# Autodesk Inventor assembly: L_Unit_SR-O
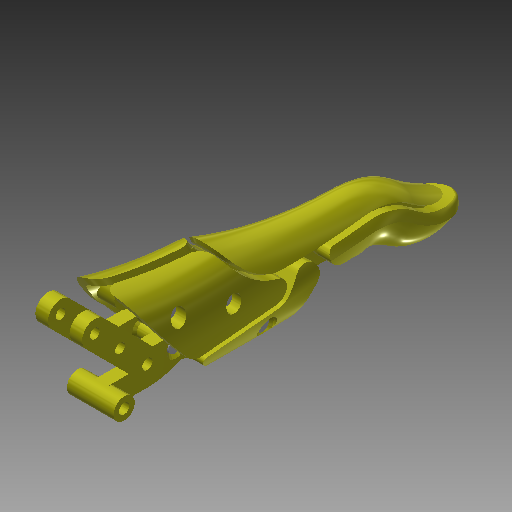
[picture p0: Inventor's stored thumbnail of the model, 512x512]
Saved by Autodesk Inventor 2018.3 (Build 223284000, 284)
## iProperties
Created: 2018-02-15
Part Number: L_Unit_SR-O
Material: 一般
Document SubType Name: Assembly
Designer: sktom
Title: Unit_SR-O
Author: sktom
## Documents named in this file (9)
- D:\CloudStrage\OneDrive\CADMech\HbSizeSMech\UnitHand\Unit_SR-H\Unit_SR-O\L_Unit_SR-O.iam
- D:\CloudStrage\OneDrive\CADMech\HbSizeSMech\UnitHand\Unit_SR-H\Unit_SR-O\L_Dummy_JointPosiion.ipt
- D:\CloudStrage\OneDrive\CADMech\HbSizeSMech\UnitHand\Unit_SR-H\Unit_SR-O\L_SR-O-01.ipt
- D:\CloudStrage\OneDrive\CADMech\HbSizeSMech\UnitHand\Unit_SR-H\Unit_SR-O\L_SR-O-02.ipt
- D:\CloudStrage\OneDrive\CADMech\HbSizeSMech\UnitHand\Unit_SR-H\Unit_SR-O\L_SR-O-03.ipt
- D:\CloudStrage\OneDrive\CADMech\HbSizeSMech\UnitHand\Unit_SR-H\Unit_SR-O\L_SR-O-04.ipt
- D:\CloudStrage\OneDrive\CADMech\HbSizeSMech\UnitHand\Unit_SR-H\Unit_SR-O\L_SR-O-05.ipt
- D:\CloudStrage\OneDrive\CADMech\HbSizeSMech\UnitHand\Unit_SR-H\Unit_SR-O\L_Parts_Shaft_Phi1.5_L6.ipt
- D:\CloudStrage\OneDrive\CADMech\HbSizeSMech\UnitHand\Unit_SR-H\Unit_SR-O\L_Parts_Screw_M1.4_L6.ipt
## Components (12 placed, 8 different names)
1. L_Dummy_JointPosiion:1 — 円柱状:3, 回転:1
2. L_SR-O-01:1 — 挿入:5, 挿入:6, 円柱状:1, 円柱状:2
3. L_SR-O-02:1 — 挿入:6, 挿入:8, 挿入:7, 回転:1
4. L_SR-O-03:1 — 挿入:2, 挿入:1, 挿入:5
5. L_SR-O-04:1 — 挿入:2, 挿入:1, 挿入:3, 挿入:4, 円柱状:3
6. L_SR-O-05:1 — 挿入:8, 挿入:7, 挿入:9, 挿入:10
7. L_Parts_Shaft_Phi1.5_L6:1 — 円柱状:1
8. L_Parts_Shaft_Phi1.5_L6:2 — 円柱状:2
9. L_Parts_Screw_M1.4_L6:1 — 挿入:4
10. L_Parts_Screw_M1.4_L6:2 — 挿入:3
11. L_Parts_Screw_M1.4_L6:3 — 挿入:9
12. L_Parts_Screw_M1.4_L6:4 — 挿入:10
## Relationships (14: Insert 10, CylindricalJoint 3, RevoluteJoint 1)
- 挿入:2 [Insert]: L_SR-O-03:1 ↔ L_SR-O-04:1
- 挿入:1 [Insert]: L_SR-O-03:1 ↔ L_SR-O-04:1
- 挿入:3 [Insert]: L_SR-O-04:1 ↔ L_Parts_Screw_M1.4_L6:2
- 挿入:4 [Insert]: L_SR-O-04:1 ↔ L_Parts_Screw_M1.4_L6:1
- 挿入:5 [Insert] (0.079 mm): L_SR-O-01:1 ↔ L_SR-O-03:1
- 挿入:6 [Insert] (0.079 mm): L_SR-O-01:1 ↔ L_SR-O-02:1
- 挿入:8 [Insert]: L_SR-O-02:1 ↔ L_SR-O-05:1
- 挿入:7 [Insert]: L_SR-O-02:1 ↔ L_SR-O-05:1
- 挿入:9 [Insert]: L_SR-O-05:1 ↔ L_Parts_Screw_M1.4_L6:3
- 挿入:10 [Insert]: L_SR-O-05:1 ↔ L_Parts_Screw_M1.4_L6:4
- 円柱状:1 [CylindricalJoint]: L_SR-O-01:1 ↔ L_Parts_Shaft_Phi1.5_L6:1
- 円柱状:2 [CylindricalJoint]: L_SR-O-01:1 ↔ L_Parts_Shaft_Phi1.5_L6:2
- 円柱状:3 [CylindricalJoint]: L_Dummy_JointPosiion:1 ↔ L_SR-O-04:1
- 回転:1 [RevoluteJoint]: L_Dummy_JointPosiion:1 ↔ L_SR-O-02:1
